# Autodesk Inventor assembly: FocusAssemblyOld
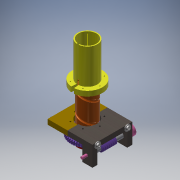
[picture p0: Inventor's stored thumbnail of the model, 180x180]
Saved by Autodesk Inventor 2019.3 (Build 233278000, 278)
## iProperties
Created: 2018-12-30
Part Number: FocusAssemblyOld
Document SubType Name: Assembly
Designer: steele
Author: steele
## Documents named in this file (10)
- C:\git\CAD-Development\robSteele\ShapeWays\TelescopeProjects\Focuser\FocusAssemblyOld.iam
- C:\git\CAD-Development\robSteele\ShapeWays\TelescopeProjects\Focuser\InnerThreadedFocusTube.ipt
- C:\git\CAD-Development\robSteele\ShapeWays\TelescopeProjects\Focuser\ExternalStationaryOuterRing.ipt
- C:\git\CAD-Development\robSteele\ShapeWays\TelescopeProjects\Focuser\ExternalMotorizedOuterRingAssembly.iam
- C:\git\CAD-Development\robSteele\ShapeWays\TelescopeProjects\Focuser\ShaftForWormGear.ipt
- C:\git\CAD-Development\robSteele\ShapeWays\TelescopeProjects\Focuser\SupportForAxel.ipt
- C:\git\CAD-Development\robSteele\ShapeWays\TelescopeProjects\Focuser\WormSpacer.ipt
- C:\git\CAD-Development\robSteele\ShapeWays\TelescopeProjects\Focuser\BottomOfSupportForAxel.ipt
- C:\git\CAD-Development\robSteele\ShapeWays\TelescopeProjects\Focuser\FocusAssembly\Design Accelerator\Bolted Connection3.iam
- c:\git\CAD-MfgResources\McMaster-Carr\BrassHeatSetInsertForPlastic\1_4-20_ 0_500 94459A390_BRASS HEAT-SET INSERT FOR PLASTIC.ipt
## Components (11 placed, 9 different names)
1. InnerThreadedFocusTube:1 — Mate:2, Flush:2, Mate:3, Insert:1
2. ExternalStationaryOuterRing:1 — Mate:2, Flush:2, Mate:3, Insert:3, Flush:5, Insert:6
3. ExternalMotorizedOuterRingAssembly:1 [sub-assembly] — Insert:1, Insert:2
4. ShaftForWormGear:1 — Insert:2, Flush:3
5. SupportForAxel:1 — Flush:3, Insert:3, Insert:4, Insert:5, Mate:6, Mate:7
6. WormSpacer:1 — Insert:4
7. WormSpacer:2 — Insert:5
8. BottomOfSupportForAxel:1 — Flush:5, Insert:6, Insert:13, Insert:14
9. 1_4-20_ 0_500 94459A390_BRASS HEAT-SET INSERT FOR PLASTIC:1 — Insert:14
10. 1_4-20_ 0_500 94459A390_BRASS HEAT-SET INSERT FOR PLASTIC:2 — Insert:13
11. Bolted Connection:2 [sub-assembly] — Mate:6, Mate:7
## Relationships (15: Insert 8, Mate 4, Flush 3)
- Mate:2: InnerThreadedFocusTube:1 ↔ ExternalStationaryOuterRing:1
- Flush:2: InnerThreadedFocusTube:1 ↔ ExternalStationaryOuterRing:1
- Mate:3: InnerThreadedFocusTube:1 ↔ ExternalStationaryOuterRing:1
- Insert:1: InnerThreadedFocusTube:1 ↔ ExternalMotorizedOuterRingAssembly:1
- Insert:2 (44.45 mm): ExternalMotorizedOuterRingAssembly:1 ↔ ShaftForWormGear:1
- Flush:3: ShaftForWormGear:1 ↔ SupportForAxel:1
- Insert:3 (76.2 mm): ExternalStationaryOuterRing:1 ↔ SupportForAxel:1
- Insert:4 (0.254 mm): SupportForAxel:1 ↔ WormSpacer:1
- Insert:5 (0.254 mm): SupportForAxel:1 ↔ WormSpacer:2
- Flush:5: ExternalStationaryOuterRing:1 ↔ BottomOfSupportForAxel:1
- Insert:6 (-76.2 mm): ExternalStationaryOuterRing:1 ↔ BottomOfSupportForAxel:1
- Insert:13: BottomOfSupportForAxel:1 ↔ 1_4-20_ 0_500 94459A390_BRASS HEAT-SET INSERT FOR PLASTIC:2
- Insert:14: BottomOfSupportForAxel:1 ↔ 1_4-20_ 0_500 94459A390_BRASS HEAT-SET INSERT FOR PLASTIC:1
- Mate:6: SupportForAxel:1 ↔ Bolted Connection:2
- Mate:7: SupportForAxel:1 ↔ Bolted Connection:2
